# Autodesk Inventor assembly: Rev extrusion 90 degree test
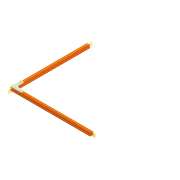
[picture p0: Inventor's stored thumbnail of the model, 180x180]
Saved by Autodesk Inventor 2020 (Build 240168000, 168)
## iProperties
Created: 2019-11-22
Part Number: Rev extrusion 90 degree test
Document SubType Name: Assembly
Designer: ball
Author: ball
## Documents named in this file (4)
- C:\FTC\FTC8863CAD\2019 Robot\Delivery\Rev extrusion 90 degree test.iam
- C:\FTC\FTC8863CAD\RevRobotics\REV-41-1017_15mm_extrusion_17.875in.ipt
- C:\FTC\FTC8863CAD\RevRobotics\REV-41-1305 90 degree plastic bracket.ipt
- C:\FTC\FTC8863CAD\StepLibraries\Nuts\m3 18-8 STAINLESS STL NYLON-INSERT LOCKNUT.ipt
## Components (4 placed, 3 different names)
1. REV-41-1017_15mm_extrusion_17.875in:1 — Mate:1, Flush:1, Flush:2, Flush:4
2. REV-41-1017_15mm_extrusion_17.875in:2 — Mate:1, Flush:1, Flush:2, Mate:2, Flush:3
3. REV-41-1305 90 degree plastic bracket:1 — Mate:2, Flush:3, Flush:4, Mate:3, Mate:4
4. m3 18-8 STAINLESS STL NYLON-INSERT LOCKNUT:1 — Mate:3, Mate:4
## Relationships (8: Mate 4, Flush 4)
- Mate:1: REV-41-1017_15mm_extrusion_17.875in:1 ↔ REV-41-1017_15mm_extrusion_17.875in:2
- Flush:1: REV-41-1017_15mm_extrusion_17.875in:1 ↔ REV-41-1017_15mm_extrusion_17.875in:2
- Flush:2: REV-41-1017_15mm_extrusion_17.875in:1 ↔ REV-41-1017_15mm_extrusion_17.875in:2
- Mate:2: REV-41-1017_15mm_extrusion_17.875in:2 ↔ REV-41-1305 90 degree plastic bracket:1
- Flush:3: REV-41-1017_15mm_extrusion_17.875in:2 ↔ REV-41-1305 90 degree plastic bracket:1
- Flush:4: REV-41-1017_15mm_extrusion_17.875in:1 ↔ REV-41-1305 90 degree plastic bracket:1
- Mate:3: REV-41-1305 90 degree plastic bracket:1 ↔ m3 18-8 STAINLESS STL NYLON-INSERT LOCKNUT:1
- Mate:4: REV-41-1305 90 degree plastic bracket:1 ↔ m3 18-8 STAINLESS STL NYLON-INSERT LOCKNUT:1
